# Autodesk Inventor assembly: Ensamble_5
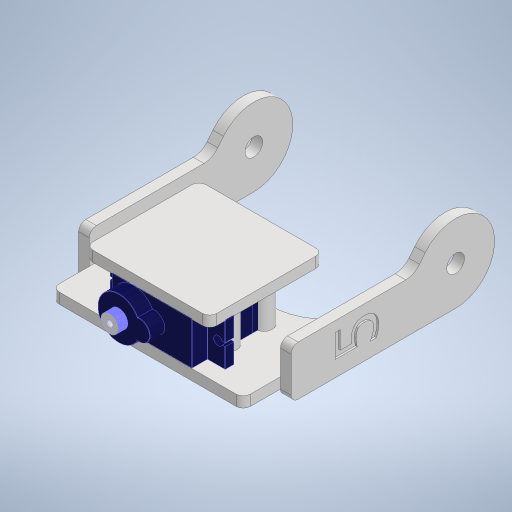
[picture p0: Inventor's stored thumbnail of the model, 512x512]
Saved by Autodesk Inventor 2023 (Build 270158000, 158)
## iProperties
Created: 2024-09-27
Part Number: Ensamble_5
Document SubType Name: Assembly
Designer: sebas
Author: sebas
## Documents named in this file (3)
- C:\Users\sebas\OneDrive\Documentos\ILLERO_MODELADO_ROBOT\Ensamble_5.iam
- C:\Users\sebas\OneDrive\Documentos\ILLERO_MODELADO_ROBOT\Pieza_5.ipt
- C:\Users\sebas\OneDrive\Documentos\ILLERO_MODELADO_ROBOT\MicroServo-SG90.ipt
## Components (2 placed, 2 different names)
1. Pieza_5:1 — Coincidencia:34, Nivelación:1, Nivelación:2, Coincidencia:35, Nivelación:3
2. MicroServo-SG90:1 — Coincidencia:34, Nivelación:1, Nivelación:2
## Relationships (5: Flush 3, Mate 2)
- Coincidencia:34 [Mate]: Pieza_5:1 ↔ MicroServo-SG90:1
- Nivelación:1 [Flush]: Pieza_5:1 ↔ MicroServo-SG90:1
- Nivelación:2 [Flush]: Pieza_5:1 ↔ MicroServo-SG90:1
- Coincidencia:35 [Mate]: Pieza_5:1
- Nivelación:3 [Flush]: Pieza_5:1
